# Autodesk Inventor assembly: Assembly2
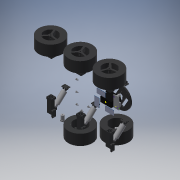
[picture p0: Inventor's stored thumbnail of the model, 180x180]
Saved by Autodesk Inventor 2016 (Build 200138000, 138)
## iProperties
Created: 2015-06-07
Part Number: Assembly2
Document SubType Name: Assembly
Designer: Jufo
Author: Jufo
## Documents named in this file (31)
- C:\Users\Juraj\Documents\GitHub\Robot6x6\Terrenny robot CAD\Assembly2.iam
- C:\Users\Juraj\Documents\GitHub\Robot6x6\Terrenny robot CAD\Part1.ipt
- C:\Users\Juraj\Documents\GitHub\Robot6x6\Terrenny robot CAD\Part2.ipt
- C:\Users\Juraj\Documents\GitHub\Robot6x6\Terrenny robot CAD\Part3.ipt
- C:\Users\Juraj\Documents\GitHub\Robot6x6\Terrenny robot CAD\motoruchyt.ipt
- C:\Users\Juraj\Documents\GitHub\Robot6x6\Terrenny robot CAD\Part1 (2).ipt
- C:\Users\Juraj\Documents\GitHub\Robot6x6\Terrenny robot CAD\pruzina.ipt
- C:\Users\Juraj\Documents\GitHub\Robot6x6\Terrenny robot CAD\koleso.ipt
- C:\Users\Juraj\Documents\GitHub\Robot6x6\Terrenny robot CAD\Kinect\kinect assembly.iam
- C:\Users\Juraj\Documents\GitHub\Robot6x6\Terrenny robot CAD\bateria.ipt
- C:\Users\Juraj\Documents\GitHub\Robot6x6\Terrenny robot CAD\M3x6.ipt
- C:\Users\Juraj\Documents\GitHub\Robot6x6\Terrenny robot CAD\raspberry-pi-2-model-b-3d-cad-assembly-model-2.snapshot.18\Imported Components\RaspberryPi2 STEP214\RaspberryPi2 STEP214.iam
- C:\Users\Juraj\Documents\GitHub\Robot6x6\Terrenny robot CAD\Part37.ipt
- C:\Users\Juraj\Documents\GitHub\Robot6x6\Terrenny robot CAD\vrch1.ipt
- C:\Users\Juraj\Documents\GitHub\Robot6x6\Terrenny robot CAD\vrch2.ipt
- C:\Users\Juraj\Documents\GitHub\Robot6x6\Terrenny robot CAD\mg996r-servo.snapshot.1\MG996R\Imported Components\MG996R\MG996R.iam
- C:\Users\Juraj\Documents\GitHub\Robot6x6\Terrenny robot CAD\kinectUchyt.ipt
- C:\Users\Juraj\Documents\GitHub\Robot6x6\Terrenny robot CAD\arduino-l298n-1.snapshot.1\L298N.ipt
- C:\Users\Juraj\Documents\GitHub\Robot6x6\Terrenny robot CAD\router.ipt
- C:\Users\Juraj\Documents\GitHub\Robot6x6\Terrenny robot CAD\Part53.ipt
- C:\Users\Juraj\Documents\GitHub\Robot6x6\Terrenny robot CAD\DS1302.ipt
- C:\Users\Juraj\Documents\GitHub\Robot6x6\Terrenny robot CAD\relay_module.ipt
- C:\Users\Juraj\Documents\GitHub\Robot6x6\Terrenny robot CAD\DC menic.ipt
- C:\Users\Juraj\Documents\GitHub\Robot6x6\Terrenny robot CAD\wifi-antenna-1.snapshot.1\Imported Components\Antenna hub\Antenna hub.ipt
- C:\Users\Juraj\Documents\GitHub\Robot6x6\Terrenny robot CAD\wifi-antenna-1.snapshot.1\Imported Components\Antennae\Antennae.ipt
- C:\Users\Juraj\Documents\GitHub\Robot6x6\Terrenny robot CAD\tlacitko.ipt
- C:\Users\Juraj\Documents\GitHub\Robot6x6\Terrenny robot CAD\rj45.ipt
- C:\Users\Juraj\Documents\GitHub\Robot6x6\Terrenny robot CAD\GPS sensor.ipt
- C:\Users\Juraj\Documents\GitHub\Robot6x6\Terrenny robot CAD\ACS712(prudovy snimac).ipt
- C:\Users\Juraj\Documents\GitHub\Robot6x6\Terrenny robot CAD\accelerometer.ipt
- C:\Users\Juraj\Documents\GitHub\Robot6x6\Terrenny robot CAD\arduino-pro-mini-1.snapshot.4\Arduino Pro Mini\Arduino_pro_mini.ipt
## Components (72 placed, 30 different names)
1. Arduino_pro_mini:1 — Mate:63, Mate:75
2. Arduino_pro_mini:2 — Mate:74
3. Arduino_pro_mini:3 — Mate:65
4. DC menic:3 — Insert:112
5. accelerometer:1 — Mate:56
6. rj45:1 — Mate:57, Mate:58, Mate:59
7. GPS sensor:1 — Mate:60
8. tlacitko:3 — Insert:96
9. tlacitko:2 — Insert:95
10. tlacitko:1 — Insert:97
11. Antenna hub:1 — Insert:86, Insert:87
12. Antenna hub:2 — Insert:85, Insert:88
13. Antennae:2 — Insert:85
14. Antennae:1 — Insert:86
15. vrch1:1 — Insert:65, Insert:66, Insert:69, Insert:70, Mate:56
16. vrch2:1 — Insert:67, Insert:68, Insert:87, Insert:88, Mate:57, Mate:58, Mate:59, Mate:60, Insert:95, Insert:96, Insert:97
17. kinect assembly:1 [sub-assembly] — Insert:72
18. DS1302:1 — Insert:100, Insert:101
19. relay_module:1 — Insert:98, Insert:99
20. DC menic:2 — Insert:111
21. DC menic:1 — Insert:110
22. ACS712(prudovy snimac):1 — Mate:54, Mate:55
23. RaspberryPi2 STEP214:1 [sub-assembly] — Insert:102, Insert:103
24. router:1 — Mate:38
25. L298N:1 — Insert:115, Insert:116
26. L298N:2 — Insert:113, Insert:114
27. L298N:3 — Insert:117, Insert:118
28. medzicast_zadna — Insert:75, Insert:76, Mate:54, Insert:98, Insert:99, Insert:100, Insert:101, Insert:102, Insert:103
29. medzicast_predna — Mate:38, Insert:73, Insert:74, Mate:63, Mate:65, Mate:74, Mate:75, Insert:110, Insert:111, Insert:112, Insert:113, Insert:114, Insert:115, Insert:116, Insert:117, Insert:118
30. spodok_predny — Insert:1, Insert:2, Insert:3, Insert:4, Insert:5, Insert:9, Insert:10, Insert:11, Insert:13, Insert:14, Insert:29, Insert:30, Insert:31, Insert:32, Angle:1, Angle:2, Angle:4, Angle:5, Insert:65, Insert:66, Insert:73, Insert:74
31. spodok_zadny — Insert:1, Insert:6, Insert:7, Insert:8, Insert:10, Insert:12, Insert:22, Insert:28, Insert:39, Angle:3, Angle:6, Insert:56, Insert:57, Insert:58, Insert:59, Insert:60, Insert:61, Insert:67, Insert:68, Insert:75, Insert:76, Mate:41, Mate:42, Mate:43, Mate:44, Mate:45, Mate:46
32. bateria:1 — Mate:41, Mate:44, Mate:45, Mate:55
33. bateria:2 — Mate:42, Mate:43, Mate:46
34. M3x6:1 — Insert:56
35. M3x6:2 — Insert:59
36. M3x6:3 — Insert:60
37. M3x6:4 — Insert:57
38. M3x6:5 — Insert:58
39. M3x6:8
40. M3x6:9 — Insert:61
41. Part3:1 — Insert:5, Insert:23, Insert:32
42. Part3:2 — Insert:7, Insert:27, Insert:28
43. Part3:3 — Insert:6, Insert:21, Insert:22, Insert:39
44. Part3:4 — Insert:4, Insert:24, Insert:31
45. Part3:5 — Insert:3, Insert:26, Insert:29
46. Part3:6 — Insert:2, Insert:25, Insert:30
47. motoruchyt:1 — Insert:13, Insert:16
48. motoruchyt:2 — Insert:11, Insert:20
49. motoruchyt:3 — Insert:9, Insert:19
50. motoruchyt:4 — Insert:8, Insert:18
51. motoruchyt:5 — Insert:14, Insert:15
52. motoruchyt:6 — Insert:12, Insert:17
53. pruzina:1 — Insert:21
54. pruzina:2 — Insert:26
55. pruzina:3 — Insert:23
56. pruzina:4 — Insert:24
57. pruzina:5 — Insert:27
58. pruzina:6 — Insert:25
59. MG996R:1 [sub-assembly] — Insert:69, Insert:70, Insert:71
60. kinectUchyt:1 — Insert:71, Insert:72
61. Part1 (2):1 — Insert:15, Insert:34
62. Part1 (2):2 — Insert:16, Insert:38
63. Part1 (2):3 — Insert:17, Insert:35
64. Part1 (2):4 — Insert:19, Insert:33
65. Part1 (2):5 — Insert:18, Insert:36
66. Part1 (2):6 — Insert:20, Insert:37
67. koleso:1 — Insert:37, Angle:1
68. koleso:2 — Insert:38, Angle:5
69. koleso:3 — Insert:34, Angle:4
70. koleso:4 — Insert:33, Angle:2
71. koleso:5 — Insert:35, Angle:6
72. koleso:6 — Insert:36, Angle:3
## Relationships (103: Insert 79, Mate 18, Angle 6)
- Insert:1: spodok_predny ↔ spodok_zadny
- Insert:2: spodok_predny ↔ Part3:6
- Insert:3: spodok_predny ↔ Part3:5
- Insert:4: spodok_predny ↔ Part3:4
- Insert:5: spodok_predny ↔ Part3:1
- Insert:6: spodok_zadny ↔ Part3:3
- Insert:7: spodok_zadny ↔ Part3:2
- Insert:8 (0.5 mm): spodok_zadny ↔ motoruchyt:4
- Insert:9 (0.5 mm): spodok_predny ↔ motoruchyt:3
- Insert:10: spodok_predny ↔ spodok_zadny
- Insert:11 (0.5 mm): spodok_predny ↔ motoruchyt:2
- Insert:12 (0.5 mm): spodok_zadny ↔ motoruchyt:6
- Insert:13 (0.5 mm): spodok_predny ↔ motoruchyt:1
- Insert:14 (0.5 mm): spodok_predny ↔ motoruchyt:5
- Insert:15: motoruchyt:5 ↔ Part1 (2):1
- Insert:16 (2 mm): motoruchyt:1 ↔ Part1 (2):2
- Insert:17: motoruchyt:6 ↔ Part1 (2):3
- Insert:18: motoruchyt:4 ↔ Part1 (2):5
- Insert:19 (2 mm): motoruchyt:3 ↔ Part1 (2):4
- Insert:20 (2 mm): motoruchyt:2 ↔ Part1 (2):6
- Insert:21: Part3:3 ↔ pruzina:1
- Insert:22: spodok_zadny ↔ Part3:3
- Insert:23: Part3:1 ↔ pruzina:3
- Insert:24: Part3:4 ↔ pruzina:4
- Insert:25: Part3:6 ↔ pruzina:6
- Insert:26: Part3:5 ↔ pruzina:2
- Insert:27: Part3:2 ↔ pruzina:5
- Insert:28: spodok_zadny ↔ Part3:2
- Insert:29: spodok_predny ↔ Part3:5
- Insert:30: spodok_predny ↔ Part3:6
- Insert:31: spodok_predny ↔ Part3:4
- Insert:32: spodok_predny ↔ Part3:1
- Insert:33: Part1 (2):4 ↔ koleso:4
- Insert:34: Part1 (2):1 ↔ koleso:3
- Insert:35: Part1 (2):3 ↔ koleso:5
- Insert:36: Part1 (2):5 ↔ koleso:6
- Insert:37: Part1 (2):6 ↔ koleso:1
- Insert:38: Part1 (2):2 ↔ koleso:2
- Insert:39: spodok_zadny ↔ Part3:3
- Angle:1 (180 deg): spodok_predny ↔ koleso:1
- Angle:2 (180 deg): spodok_predny ↔ koleso:4
- Angle:3 (180 deg): spodok_zadny ↔ koleso:6
- Angle:4 (180 deg): spodok_predny ↔ koleso:3
- Angle:5 (180 deg): spodok_predny ↔ koleso:2
- Angle:6 (180 deg): spodok_zadny ↔ koleso:5
- Insert:56 (-6 mm): spodok_zadny ↔ M3x6:1
- Insert:57 (-6 mm): spodok_zadny ↔ M3x6:4
- Insert:58 (-6 mm): spodok_zadny ↔ M3x6:5
- Insert:59 (-6 mm): spodok_zadny ↔ M3x6:2
- Insert:60 (-6 mm): spodok_zadny ↔ M3x6:3
- Insert:61 (-6 mm): spodok_zadny ↔ M3x6:9
- Insert:65: vrch1:1 ↔ spodok_predny
- Insert:66: vrch1:1 ↔ spodok_predny
- Insert:67: vrch2:1 ↔ spodok_zadny
- Insert:68: vrch2:1 ↔ spodok_zadny
- Insert:69: vrch1:1 ↔ MG996R:1
- Insert:70: vrch1:1 ↔ MG996R:1
- Insert:71: MG996R:1 ↔ kinectUchyt:1
- Mate:38: router:1 ↔ medzicast_predna
- Insert:72: kinect assembly:1 ↔ kinectUchyt:1
- Insert:73: medzicast_predna ↔ spodok_predny
- Insert:74: medzicast_predna ↔ spodok_predny
- Insert:75: medzicast_zadna ↔ spodok_zadny
- Insert:76: medzicast_zadna ↔ spodok_zadny
- Mate:41: spodok_zadny ↔ bateria:1
- Mate:42: spodok_zadny ↔ bateria:2
- Mate:43 (1 mm): spodok_zadny ↔ bateria:2
- Mate:44 (1 mm): spodok_zadny ↔ bateria:1
- Mate:45 (1 mm): spodok_zadny ↔ bateria:1
- Mate:46: spodok_zadny ↔ bateria:2
- Insert:85: Antenna hub:2 ↔ Antennae:2
- Insert:86: Antenna hub:1 ↔ Antennae:1
- Insert:87: Antenna hub:1 ↔ vrch2:1
- Insert:88: Antenna hub:2 ↔ vrch2:1
- Mate:54: ACS712(prudovy snimac):1 ↔ medzicast_zadna
- Mate:55 (20 mm): ACS712(prudovy snimac):1 ↔ bateria:1
- Mate:56: accelerometer:1 ↔ vrch1:1
- Mate:57 (-4 mm): rj45:1 ↔ vrch2:1
- Mate:58 (0.5 mm): rj45:1 ↔ vrch2:1
- Mate:59 (0.5 mm): rj45:1 ↔ vrch2:1
- Mate:60 (0.3 mm): GPS sensor:1 ↔ vrch2:1
- Insert:95: tlacitko:2 ↔ vrch2:1
- Insert:96: tlacitko:3 ↔ vrch2:1
- Insert:97: tlacitko:1 ↔ vrch2:1
- Insert:98: relay_module:1 ↔ medzicast_zadna
- Insert:99: relay_module:1 ↔ medzicast_zadna
- Insert:100: DS1302:1 ↔ medzicast_zadna
- Insert:101: DS1302:1 ↔ medzicast_zadna
- Insert:102: RaspberryPi2 STEP214:1 ↔ medzicast_zadna
- Insert:103: RaspberryPi2 STEP214:1 ↔ medzicast_zadna
- Mate:63: Arduino_pro_mini:1 ↔ medzicast_predna
- Mate:65: Arduino_pro_mini:3 ↔ medzicast_predna
- Mate:74: Arduino_pro_mini:2 ↔ medzicast_predna
- Mate:75 (55 mm): Arduino_pro_mini:1 ↔ medzicast_predna
- Insert:110: DC menic:1 ↔ medzicast_predna
- Insert:111: DC menic:2 ↔ medzicast_predna
- Insert:112: DC menic:3 ↔ medzicast_predna
- Insert:113: L298N:2 ↔ medzicast_predna
- Insert:114: L298N:2 ↔ medzicast_predna
- Insert:115: L298N:1 ↔ medzicast_predna
- Insert:116: L298N:1 ↔ medzicast_predna
- Insert:117: L298N:3 ↔ medzicast_predna
- Insert:118: L298N:3 ↔ medzicast_predna
